# Autodesk Inventor assembly: Gripper_assembly
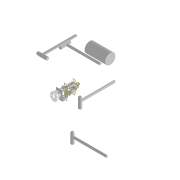
[picture p0: Inventor's stored thumbnail of the model, 180x180]
Saved by Autodesk Inventor 2022 (Build 260153000, 153)
## iProperties
Created: 2022-08-27
Part Number: Gripper_assembly
Document SubType Name: Assembly
Designer: dell
Author: dell
## Documents named in this file (10)
- D:\xxxx\Uni\Part IV\MECHENG_736\Gripper_project\Gripper_assembly.iam
- D:\xxxx\Uni\Part IV\MECHENG_736\Gripper_project\dovetail_female.ipt
- D:\xxxx\Uni\Part IV\MECHENG_736\Gripper_project\XM430.iam
- D:\xxxx\Uni\Part IV\MECHENG_736\Gripper_project\Mount_UR.ipt
- D:\xxxx\Uni\Part IV\MECHENG_736\Gripper_project\Motor_pulley.ipt
- D:\xxxx\Uni\Part IV\MECHENG_736\Gripper_project\Motor_plate.ipt
- D:\xxxx\Uni\Part IV\MECHENG_736\Gripper_project\Proximal_phalange.ipt
- D:\xxxx\Uni\Part IV\MECHENG_736\Gripper_project\Middle_phalange.ipt
- D:\xxxx\Uni\Part IV\MECHENG_736\Gripper_project\Hammer.ipt
- D:\xxxx\Uni\Part IV\MECHENG_736\Gripper_project\1.5L_Bottle.ipt
## Components (14 placed, 9 different names)
1. dovetail_female:1 — Mate:1, Mate:2, Flush:1, Mate:3, Mate:4
2. XM430:2 [sub-assembly] — Flush:1, Mate:3, Mate:4, Mate:6, Mate:7, Mate:8, Mate:9, Mate:18
3. Mount_UR:1 — Mate:1, Mate:2
4. Motor_pulley:1 — Mate:6, Mate:18
5. Motor_plate:1 — Mate:7, Mate:8, Mate:9, Mate:10, Mate:11, Angle:2, Mate:14, Mate:15, Angle:3
6. Proximal_phalange:1 — Mate:10, Mate:11, Mate:12, Mate:13, Angle:2
7. Middle_phalange:1 — Mate:12, Mate:13
8. Hammer:1
9. Hammer:2
10. Hammer:3
11. Proximal_phalange:3 — Mate:14, Mate:15, Mate:16, Mate:17, Angle:3
12. Middle_phalange:4 — Mate:16, Mate:17
13. Hammer:4
14. 1.5L_Bottle:1
## Relationships (20: Mate 17, Angle 2, Flush 1)
- Mate:1: dovetail_female:1 ↔ Mount_UR:1
- Mate:2: dovetail_female:1 ↔ Mount_UR:1
- Flush:1: dovetail_female:1 ↔ XM430:2
- Mate:3: dovetail_female:1 ↔ XM430:2
- Mate:4: dovetail_female:1 ↔ XM430:2
- Mate:6: XM430:2 ↔ Motor_pulley:1
- Mate:7: XM430:2 ↔ Motor_plate:1
- Mate:8: XM430:2 ↔ Motor_plate:1
- Mate:9: XM430:2 ↔ Motor_plate:1
- Mate:10: Motor_plate:1 ↔ Proximal_phalange:1
- Mate:11: Motor_plate:1 ↔ Proximal_phalange:1
- Mate:12: Proximal_phalange:1 ↔ Middle_phalange:1
- Mate:13: Proximal_phalange:1 ↔ Middle_phalange:1
- Angle:2 (90 deg): Motor_plate:1 ↔ Proximal_phalange:1
- Mate:14: Motor_plate:1 ↔ Proximal_phalange:3
- Mate:15: Motor_plate:1 ↔ Proximal_phalange:3
- Mate:16: Proximal_phalange:3 ↔ Middle_phalange:4
- Mate:17: Proximal_phalange:3 ↔ Middle_phalange:4
- Angle:3 (100 deg): Motor_plate:1 ↔ Proximal_phalange:3
- Mate:18: XM430:2 ↔ Motor_pulley:1
